# Autodesk Inventor assembly: 스카치 요크
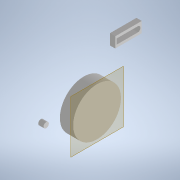
[picture p0: Inventor's stored thumbnail of the model, 180x180]
Saved by Autodesk Inventor 2022 (Build 260153000, 153)
## iProperties
Created: 2022-10-28
Part Number: 스카치 요크
Document SubType Name: Assembly
Designer: gogin
Author: gogin
## Documents named in this file (4)
- C:\Users\gogin\Desktop\대학교\SIor\스카치 요크.iam
- C:\Users\gogin\Desktop\대학교\SIor\작은 원통.ipt
- C:\Users\gogin\Desktop\대학교\SIor\큰 원통.ipt
- C:\Users\gogin\Desktop\대학교\SIor\뚫린 직육면체.ipt
## Components (3 placed, 3 different names)
1. 작은 원통:1 — 플러쉬:1
2. 큰 원통:1 — 플러쉬:1
3. 뚫린 직육면체:1
## Relationships (1: Flush 1)
- 플러쉬:1 [Flush]: 작은 원통:1 ↔ 큰 원통:1
